# Autodesk Inventor assembly: iot-ball
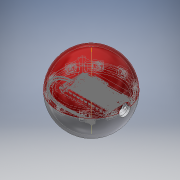
[picture p0: Inventor's stored thumbnail of the model, 180x180]
Saved by Autodesk Inventor 2018 (Build 220112000, 112)
## iProperties
Created: 2018-04-12
Part Number: iot-ball
Document SubType Name: Assembly
Designer: Raghava
Author: Raghava
## Documents named in this file (5)
- C:\Users\Raghava\Desktop\iot-ball\cad\iot-ball.iam
- C:\Users\Raghava\Desktop\iot-ball\cad\lattice-ball-bottom.ipt
- C:\Users\Raghava\Desktop\iot-ball\cad\lattice-ball-top.ipt
- C:\Users\Raghava\Desktop\iot-ball\cad\electronics-subassembly.iam
- C:\Users\Raghava\Desktop\iot-ball\cad\neopixel-minipcb.iam
## Components (13 placed, 4 different names)
1. lattice-ball-bottom:1 — Mate:1, Mate:3, Mate:4, Mate:5
2. lattice-ball-top:1 — Mate:3
3. electronics-subassembly:1 [sub-assembly] — Mate:4
4. neopixel-minipcb:1 [sub-assembly] — Mate:5
5. neopixel-minipcb:2 [sub-assembly]
6. neopixel-minipcb:3 [sub-assembly]
7. neopixel-minipcb:4 [sub-assembly]
8. neopixel-minipcb:5 [sub-assembly]
9. neopixel-minipcb:6 [sub-assembly]
10. neopixel-minipcb:7 [sub-assembly]
11. neopixel-minipcb:8 [sub-assembly]
12. neopixel-minipcb:9 [sub-assembly]
13. neopixel-minipcb:10 [sub-assembly]
## Component patterns: (10 elements, first: neopixel-minipcb:1)
## Relationships (4: Mate 4)
- Mate:1: lattice-ball-bottom:1
- Mate:3: lattice-ball-bottom:1 ↔ lattice-ball-top:1
- Mate:4: lattice-ball-bottom:1 ↔ electronics-subassembly:1
- Mate:5: lattice-ball-bottom:1 ↔ neopixel-minipcb:1
